# Autodesk Inventor assembly: Сборка3
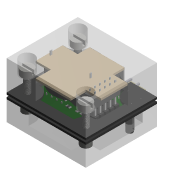
[picture p0: Inventor's stored thumbnail of the model, 180x180]
Saved by Autodesk Inventor 2015 SP1 (Build 190203100, 203)
## iProperties
Created: 2015-12-01
Part Number: Сборка3
Document SubType Name: Assembly
Designer: User
Mass: 33.0279 g
Surface Area: 226.442 cm^2
Volume: 24.1057 cm^3
Density: 1.37013 g/cm^3
Author: User
Title: external
## Documents named in this file (12)
- C:\Users\User\Downloads\kurs_mark\Inventor\ext.iam
- C:\Users\User\Downloads\kurs_mark\Inventor\conn_sensor.ipt
- C:\Users\User\Downloads\kurs_mark\Inventor\button.ipt
- C:\Users\User\Downloads\kurs_mark\Inventor\Imported Components\fuel_level_1h2\fuel_level_1h2.iam
- C:\Users\User\Downloads\kurs_mark\Inventor\case_top.ipt
- C:\Users\User\Downloads\kurs_mark\Inventor\hdr-2x5t_2.54x2.54_13x5.ipt
- C:\Users\User\Downloads\kurs_mark\Inventor\case_bottom.ipt
- C:\Users\User\Downloads\kurs_mark\Inventor\resin_bottom.ipt
- C:\Users\User\Downloads\kurs_mark\Inventor\resin_top.ipt
- C:\Users\User\Downloads\kurs_mark\Inventor\bonka.ipt
- C:\Users\User\Downloads\kurs_mark\Inventor\screw_M3-16.ipt
- C:\Users\User\Downloads\kurs_mark\Inventor\pcb_btm.iam
## Components (15 placed, 11 different names)
1. conn_sensor:1 — Жесткий:2
2. button:1 — Жесткий:3
3. fuel_level_1h2:1 [sub-assembly] — Жесткий:2, Жесткий:3, Заподлицо:3
4. case_top:1 — Цилиндрический:1, Жесткий:6, Rigid:7, Rigid:8, Rigid:9
5. hdr-2x5t_2.54x2.54_13x5:1
6. case_bottom:1 — Цилиндрический:1, Rigid:10, Rigid:11, Rigid:12, Совмещение:1, Совмещение:2, Совмещение:3
7. resin_bottom:1
8. resin_top:1 — Жесткий:6
9. bonka:1 — Rigid:7
10. bonka:2 — Rigid:8
11. bonka:3 — Rigid:9
12. screw_M3-16:1 — Rigid:12
13. screw_M3-16:2 — Rigid:11
14. screw_M3-16:3 — Rigid:10
15. pcb_btm:1 [sub-assembly] — Совмещение:1, Совмещение:2, Совмещение:3
## Relationships (14: WeldJoint 9, Mate 3, Flush 1, CylindricalJoint 1)
- Жесткий:2 [WeldJoint] (0.3 mm): conn_sensor:1 ↔ fuel_level_1h2:1
- Жесткий:3 [WeldJoint]: button:1 ↔ fuel_level_1h2:1
- Заподлицо:3 [Flush]: fuel_level_1h2:1
- Цилиндрический:1 [CylindricalJoint]: case_top:1 ↔ case_bottom:1
- Жесткий:6 [WeldJoint]: case_top:1 ↔ resin_top:1
- Rigid:7 [WeldJoint]: case_top:1 ↔ bonka:1
- Rigid:8 [WeldJoint]: case_top:1 ↔ bonka:2
- Rigid:9 [WeldJoint]: case_top:1 ↔ bonka:3
- Rigid:10 [WeldJoint]: case_bottom:1 ↔ screw_M3-16:3
- Rigid:11 [WeldJoint]: case_bottom:1 ↔ screw_M3-16:2
- Rigid:12 [WeldJoint]: case_bottom:1 ↔ screw_M3-16:1
- Совмещение:1 [Mate]: case_bottom:1 ↔ pcb_btm:1
- Совмещение:2 [Mate]: case_bottom:1 ↔ pcb_btm:1
- Совмещение:3 [Mate]: case_bottom:1 ↔ pcb_btm:1
